# Autodesk Inventor assembly: electronics_v2
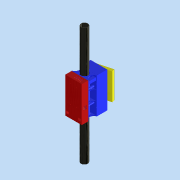
[picture p0: Inventor's stored thumbnail of the model, 180x180]
Saved by Autodesk Inventor 2022 (Build 260153000, 153)
## iProperties
Created: 2021-10-07
Part Number: electronics_v2
Document SubType Name: Assembly
Designer: nnico
Author: nnico
## Documents named in this file (14)
- C:\Users\nnico\Documents\Desminado Humanitario\Repositories\gpr20_electronics_box\assemblies\electronics_box.iam
- C:\Users\nnico\Documents\Desminado Humanitario\Repositories\gpr20_electronics_box\ipt\power_supply_case.ipt
- C:\Users\nnico\Documents\Desminado Humanitario\Repositories\gpr20_electronics_box\ipt\lower_pvc_adapter.ipt
- C:\Users\nnico\Documents\Desminado Humanitario\Repositories\gpr20_electronics_box\ipt\upper_pvc_adapter.ipt
- C:\Users\nnico\Documents\Desminado Humanitario\Repositories\gpr20_electronics_box\ipt\electronics_case.ipt
- C:\Users\nnico\Documents\Desminado Humanitario\Repositories\gpr20_electronics_box\ipt\electronics_board_tray.ipt
- C:\Users\nnico\Documents\Desminado Humanitario\Repositories\gpr20_electronics_box\ipt\raspi_board_tray.ipt
- C:\Users\nnico\Documents\Desminado Humanitario\Repositories\gpr20_electronics_box\ipt\touchscreen_support.ipt
- C:\Users\nnico\Documents\Desminado Humanitario\Repositories\gpr20_electronics_box\ipt\touchscreen_case.ipt
- C:\Users\nnico\Documents\Desminado Humanitario\Repositories\gpr20_electronics_box\ipt\touchscreen_lid.ipt
- C:\Users\nnico\Documents\Desminado Humanitario\Repositories\gpr20_electronics_box\assemblies\misc\2inx100cm_pipe.ipt
- C:\Users\nnico\Documents\Desminado Humanitario\Repositories\gpr20_electronics_box\assemblies\misc\SCREEN.ipt
- C:\Users\nnico\Documents\Desminado Humanitario\Repositories\gpr20_electronics_box\ipt\electronics_case_panel.ipt
- C:\Users\nnico\Documents\Desminado Humanitario\Repositories\gpr20_electronics_box\assemblies\misc\MEANWELL_LRS_350.ipt
## Components (13 placed, 13 different names)
1. power_supply_case:1 — Rigid:1, Rigid:11
2. lower_pvc_adapter:1 — Rigid:1, Rigid:2, Mate:1
3. upper_pvc_adapter:1 — Rigid:2, Rigid:5, Flush:1
4. electronics_case:1 — Rigid:4, Rigid:5, Rigid:6, Rigid:10
5. electronics_board_tray:1 — Rigid:3, Rigid:4
6. raspi_board_tray:1 — Rigid:3
7. touchscreen_support:1 — Rigid:6, Rigid:7
8. touchscreen_case:1 — Rigid:7, Rigid:8
9. touchscreen_lid:1 — Rigid:8, Rigid:9
10. 2inx100cm_pipe:1 — Mate:1, Flush:1
11. SCREEN:1 — Rigid:9
12. electronics_case_panel:1 — Rigid:10
13. MEANWELL_LRS_350:1 — Rigid:11
## Relationships (13: WeldJoint 11, Mate 1, Flush 1)
- Rigid:1 [WeldJoint]: power_supply_case:1 ↔ lower_pvc_adapter:1
- Rigid:2 [WeldJoint]: lower_pvc_adapter:1 ↔ upper_pvc_adapter:1
- Rigid:3 [WeldJoint]: electronics_board_tray:1 ↔ raspi_board_tray:1
- Rigid:4 [WeldJoint]: electronics_case:1 ↔ electronics_board_tray:1
- Rigid:5 [WeldJoint]: upper_pvc_adapter:1 ↔ electronics_case:1
- Rigid:6 [WeldJoint]: electronics_case:1 ↔ touchscreen_support:1
- Rigid:7 [WeldJoint]: touchscreen_support:1 ↔ touchscreen_case:1
- Rigid:8 [WeldJoint]: touchscreen_case:1 ↔ touchscreen_lid:1
- Mate:1: lower_pvc_adapter:1 ↔ 2inx100cm_pipe:1
- Flush:1 (-350 mm): upper_pvc_adapter:1 ↔ 2inx100cm_pipe:1
- Rigid:9 [WeldJoint]: touchscreen_lid:1 ↔ SCREEN:1
- Rigid:10 [WeldJoint]: electronics_case:1 ↔ electronics_case_panel:1
- Rigid:11 [WeldJoint]: power_supply_case:1 ↔ MEANWELL_LRS_350:1
